# Autodesk Inventor assembly: CO-0-1-BatteryCellPack
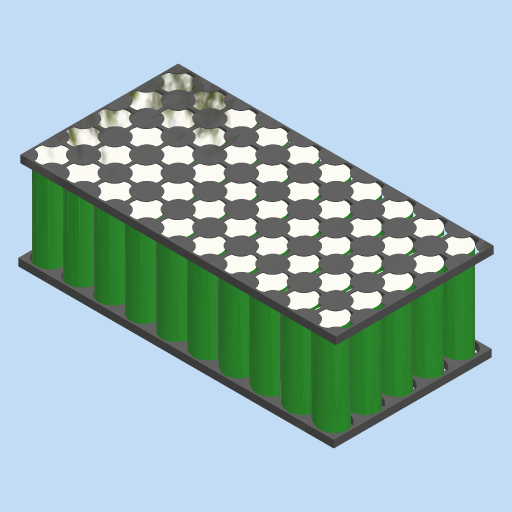
[picture p0: Inventor's stored thumbnail of the model, 512x512]
Saved by Autodesk Inventor 2023 (Build 270158000, 158)
## iProperties
Created: 2022-10-25
Part Number: CO-0-1-BatteryCellPack
Document SubType Name: Assembly
Designer: asach
Author: asach
## Documents named in this file (3)
- C:\Github\BehrendURC\CAD\Controls\CO-0-1-BatteryCellPack.iam
- C:\Github\BehrendURC\CAD\Controls\CO-1-1_CellSpacer10by5.ipt
- C:\Github\BehrendURC\CAD\Controls\CO-1-1-BatteryCell.ipt
## Components (52 placed, 2 different names)
1. CO-1-1_CellSpacer10by5:1 — Mate:2, Mate:3
2. CO-1-1_CellSpacer10by5:2 — Mate:4, Mate:5
3. CO-1-1-BatteryCell:1 — Mate:2, Mate:3, Mate:4, Mate:5
4. CO-1-1-BatteryCell:2
5. CO-1-1-BatteryCell:3
6. CO-1-1-BatteryCell:4
7. CO-1-1-BatteryCell:5
8. CO-1-1-BatteryCell:6
9. CO-1-1-BatteryCell:7
10. CO-1-1-BatteryCell:8
11. CO-1-1-BatteryCell:9
12. CO-1-1-BatteryCell:10
13. CO-1-1-BatteryCell:11
14. CO-1-1-BatteryCell:12
15. CO-1-1-BatteryCell:13
16. CO-1-1-BatteryCell:14
17. CO-1-1-BatteryCell:15
18. CO-1-1-BatteryCell:16
19. CO-1-1-BatteryCell:17
20. CO-1-1-BatteryCell:18
21. CO-1-1-BatteryCell:19
22. CO-1-1-BatteryCell:20
23. CO-1-1-BatteryCell:21
24. CO-1-1-BatteryCell:22
25. CO-1-1-BatteryCell:23
26. CO-1-1-BatteryCell:24
27. CO-1-1-BatteryCell:25
28. CO-1-1-BatteryCell:26
29. CO-1-1-BatteryCell:27
30. CO-1-1-BatteryCell:28
31. CO-1-1-BatteryCell:29
32. CO-1-1-BatteryCell:30
33. CO-1-1-BatteryCell:31
34. CO-1-1-BatteryCell:32
35. CO-1-1-BatteryCell:33
36. CO-1-1-BatteryCell:34
37. CO-1-1-BatteryCell:35
38. CO-1-1-BatteryCell:36
39. CO-1-1-BatteryCell:37
40. CO-1-1-BatteryCell:38
41. CO-1-1-BatteryCell:39
42. CO-1-1-BatteryCell:40
43. CO-1-1-BatteryCell:41
44. CO-1-1-BatteryCell:42
45. CO-1-1-BatteryCell:43
46. CO-1-1-BatteryCell:44
47. CO-1-1-BatteryCell:45
48. CO-1-1-BatteryCell:46
49. CO-1-1-BatteryCell:47
50. CO-1-1-BatteryCell:48
51. CO-1-1-BatteryCell:49
52. CO-1-1-BatteryCell:50
## Component patterns: (50 elements, first: CO-1-1-BatteryCell:1)
## Relationships (4: Mate 4)
- Mate:2: CO-1-1_CellSpacer10by5:1 ↔ CO-1-1-BatteryCell:1
- Mate:3: CO-1-1_CellSpacer10by5:1 ↔ CO-1-1-BatteryCell:1
- Mate:4: CO-1-1_CellSpacer10by5:2 ↔ CO-1-1-BatteryCell:1
- Mate:5: CO-1-1_CellSpacer10by5:2 ↔ CO-1-1-BatteryCell:1
